# Autodesk Inventor assembly: Assembly1
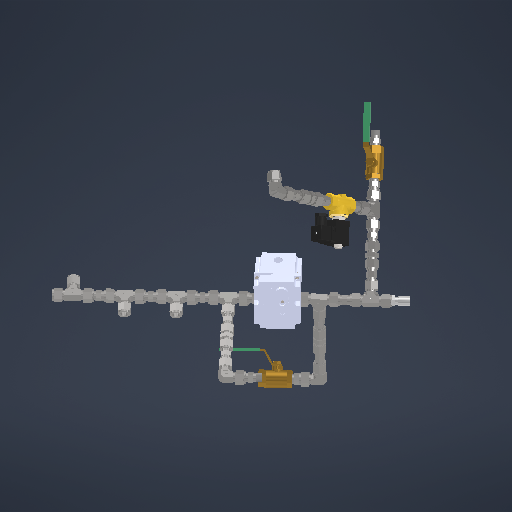
[picture p0: Inventor's stored thumbnail of the model, 512x512]
Saved by Autodesk Inventor 2026.2 (Build 302298000, 298)
## iProperties
Created: 2026-01-25
Part Number: Assembly1
Document SubType Name: Assembly
Designer: szwed
Author: szwed
## Documents named in this file (9)
- C:\Users\szwed\Desktop\R7\Assembly1.iam
- C:\Users\szwed\Documents\Inventor\Content Center Files\R2026\en-US\ISO 49 N8\ISO 49 Hexagon Nipple N8 3_8.ipt
- C:\Users\szwed\Documents\Inventor\Content Center Files\R2026\en-US\Parker A(16)\Parker A-Lok - Fractional Tube 1_2 (4).ipt
- C:\Users\szwed\Documents\Inventor\Content Center Files\R2026\en-US\Parker A(01)\Parker A-Lok - Metric to Inch Tube 12 x 1_2.ipt
- C:\Users\szwed\Documents\Inventor\Content Center Files\R2026\en-US\Parker A-Lok - 90deg Elbow - Fractional Tube\1_2(37).ipt
- C:\Users\szwed\Desktop\gs_solidworks-master\R7_GS_1110_SERVOVALVE\R7_GS_1110_SERVOVALVE\R7_GS_1110_SERVOVALVE\R7_GS_1110_SERVOVALVE.ipt
- C:\Users\szwed\Documents\Inventor\Content Center Files\R2026\en-US\Parker XV500P\Parker Female-Female Pipe Ends XV500P XV500P-8.ipt
- C:\Users\szwed\Documents\Inventor\Content Center Files\R2026\en-US\Parker MTT 2\Parker Male Taper Thread 1_4 x 3_8.ipt
- C:\Users\szwed\Downloads\MV04_DN8_3-8 Zoll\MV04_DN8_3-8 Zoll\MV04_DN8_3-8 Zoll.ipt
## Components (38 placed, 8 different names)
1. ISO 49 Hexagon Nipple N8 3/8:1 — Rigid:1, Rigid:4
2. Parker A-Lok - Fractional Tube 1/2:1 — Rigid:1, Rigid:7, Flush:3
3. ISO 49 Hexagon Nipple N8 3/8:5 — Rigid:5
4. Parker A-Lok - Fractional Tube 1/2:2 — Rigid:4
5. ISO 49 Hexagon Nipple N8 3/8:6 — Rotational:2
6. Parker A-Lok - Fractional Tube 1/2:3 — Rigid:5, Rigid:8, Flush:2
7. ISO 49 Hexagon Nipple N8 3/8:7 — Rigid:7
8. Parker A-Lok - Fractional Tube 1/2:4 — Flush:3
9. Parker A-Lok - Metric to Inch Tube 12 x 1/2:1 — Rotational:1, Rigid:9, Flush:2
10. ISO 49 Hexagon Nipple N8 3/8:8 — Rigid:8, Rotational:1
11. ISO 49 Hexagon Nipple N8 3/8:9 — Rigid:9, Rigid:10
12. Parker A-Lok - 90° Elbow - Fractional Tube 1/2:1 — Rigid:10, Cylindrical:2, Rigid:18
13. R7_GS_1110_SERVOVALVE:1 — Rotational:2, Rotational:3
14. ISO 49 Hexagon Nipple N8 3/8:10 — Rotational:3, Rigid:14
15. Parker A-Lok - Metric to Inch Tube 12 x 1/2:2 — Flush:1
16. ISO 49 Hexagon Nipple N8 3/8:12 — Mate:1, Mate:2, Mate:3
17. ISO 49 Hexagon Nipple N8 3/8:13
18. Parker A-Lok - 90° Elbow - Fractional Tube 1/2:2 — Rigid:16
19. Parker A-Lok - Fractional Tube 1/2:5 — Rigid:14, Mate:1, Rotational:7, Mate:2, Flush:1, Mate:3
20. Parker Female-Female Pipe Ends XV500P XV500P-8:1 — Rigid:17, Cylindrical:1, Rotational:6
21. ISO 49 Hexagon Nipple N8 3/8:14 — Rigid:16, Rigid:17
22. ISO 49 Hexagon Nipple N8 3/8:15 — Cylindrical:1, Cylindrical:2, Rotational:6, Rigid:18
23. ISO 49 Hexagon Nipple N8 3/8:16 — Rotational:7
24. Parker A-Lok - Fractional Tube 1/2:6 — Rotational:8, Rigid:21
25. ISO 49 Hexagon Nipple N8 3/8:17 — Rotational:8, Rotational:9
26. Parker A-Lok - Metric to Inch Tube 12 x 1/2:3 — Rotational:9, Rotational:10
27. ISO 49 Hexagon Nipple N8 3/8:18 — Rotational:10, Rotational:14
28. Parker A-Lok - Fractional Tube 1/2:7 — Rotational:12, Rigid:22, Rotational:14
29. ISO 49 Hexagon Nipple N8 3/8:19 — Rotational:12, Rigid:20
30. Parker Female-Female Pipe Ends XV500P XV500P-8:2 — Rigid:20, Rigid:27
31. Parker Male Taper Thread 1/4 x 3/8:1 — Rigid:21
32. MV04_DN8_3-8 Zoll:1 — Rigid:23, Rigid:24
33. ISO 49 Hexagon Nipple N8 3/8:20 — Rigid:22, Rigid:23
34. ISO 49 Hexagon Nipple N8 3/8:21 — Rigid:24, Rotational:13
35. Parker A-Lok - 90° Elbow - Fractional Tube 1/2:3 — Rigid:26
36. Parker A-Lok - Metric to Inch Tube 12 x 1/2:4 — Rotational:13, Rigid:25
37. ISO 49 Hexagon Nipple N8 3/8:22 — Rigid:25, Rigid:26
38. ISO 49 Hexagon Nipple N8 3/8:23 — Rigid:27
## Relationships (45: WeldJoint 25, RevoluteJoint 12, Mate 3, Flush 3, CylindricalJoint 2)
- Rigid:1 [WeldJoint]: ISO 49 Hexagon Nipple N8 3/8:1 ↔ Parker A-Lok - Fractional Tube 1/2:1
- [WeldJoint]: ISO 49 Hexagon Nipple N8 3/8:5 ↔ Parker A-Lok - Fractional Tube 1/2:2
- [WeldJoint]: ISO 49 Hexagon Nipple N8 3/8:6 ↔ Parker A-Lok - Fractional Tube 1/2:3
- Rigid:4 [WeldJoint]: ISO 49 Hexagon Nipple N8 3/8:1 ↔ Parker A-Lok - Fractional Tube 1/2:2
- Rigid:5 [WeldJoint]: ISO 49 Hexagon Nipple N8 3/8:5 ↔ Parker A-Lok - Fractional Tube 1/2:3
- [WeldJoint]: ISO 49 Hexagon Nipple N8 3/8:7 ↔ Parker A-Lok - Fractional Tube 1/2:4
- Rigid:7 [WeldJoint]: Parker A-Lok - Fractional Tube 1/2:1 ↔ ISO 49 Hexagon Nipple N8 3/8:7
- Rigid:8 [WeldJoint]: Parker A-Lok - Fractional Tube 1/2:3 ↔ ISO 49 Hexagon Nipple N8 3/8:8
- Rotational:1 [RevoluteJoint]: Parker A-Lok - Metric to Inch Tube 12 x 1/2:1 ↔ ISO 49 Hexagon Nipple N8 3/8:8
- Rigid:9 [WeldJoint]: Parker A-Lok - Metric to Inch Tube 12 x 1/2:1 ↔ ISO 49 Hexagon Nipple N8 3/8:9
- Rigid:10 [WeldJoint]: ISO 49 Hexagon Nipple N8 3/8:9 ↔ Parker A-Lok - 90° Elbow - Fractional Tube 1/2:1
- Rotational:2 [RevoluteJoint]: ISO 49 Hexagon Nipple N8 3/8:6 ↔ R7_GS_1110_SERVOVALVE:1
- Rotational:3 [RevoluteJoint]: R7_GS_1110_SERVOVALVE:1 ↔ ISO 49 Hexagon Nipple N8 3/8:10
- [RevoluteJoint]: Parker A-Lok - Metric to Inch Tube 12 x 1/2:2 ↔ ISO 49 Hexagon Nipple N8 3/8:12
- [WeldJoint]: Parker A-Lok - Metric to Inch Tube 12 x 1/2:2 ↔ ISO 49 Hexagon Nipple N8 3/8:13
- [WeldJoint]: ISO 49 Hexagon Nipple N8 3/8:13 ↔ Parker A-Lok - 90° Elbow - Fractional Tube 1/2:2
- Rigid:14 [WeldJoint]: ISO 49 Hexagon Nipple N8 3/8:10 ↔ Parker A-Lok - Fractional Tube 1/2:5
- Rigid:16 [WeldJoint]: Parker A-Lok - 90° Elbow - Fractional Tube 1/2:2 ↔ ISO 49 Hexagon Nipple N8 3/8:14
- Rigid:17 [WeldJoint] (-3 mm): Parker Female-Female Pipe Ends XV500P XV500P-8:1 ↔ ISO 49 Hexagon Nipple N8 3/8:14
- Cylindrical:1: Parker Female-Female Pipe Ends XV500P XV500P-8:1 ↔ ISO 49 Hexagon Nipple N8 3/8:15
- Cylindrical:2: Parker A-Lok - 90° Elbow - Fractional Tube 1/2:1 ↔ ISO 49 Hexagon Nipple N8 3/8:15
- Rotational:6 [RevoluteJoint]: Parker Female-Female Pipe Ends XV500P XV500P-8:1 ↔ ISO 49 Hexagon Nipple N8 3/8:15
- Rigid:18 [WeldJoint]: Parker A-Lok - 90° Elbow - Fractional Tube 1/2:1 ↔ ISO 49 Hexagon Nipple N8 3/8:15
- Mate:1: ISO 49 Hexagon Nipple N8 3/8:12 ↔ Parker A-Lok - Fractional Tube 1/2:5
- [WeldJoint]: ISO 49 Hexagon Nipple N8 3/8:16 ↔ Parker A-Lok - Fractional Tube 1/2:6
- Rotational:7 [RevoluteJoint]: Parker A-Lok - Fractional Tube 1/2:5 ↔ ISO 49 Hexagon Nipple N8 3/8:16
- Mate:2: ISO 49 Hexagon Nipple N8 3/8:12 ↔ Parker A-Lok - Fractional Tube 1/2:5
- Flush:1: Parker A-Lok - Metric to Inch Tube 12 x 1/2:2 ↔ Parker A-Lok - Fractional Tube 1/2:5
- Rotational:8 [RevoluteJoint]: Parker A-Lok - Fractional Tube 1/2:6 ↔ ISO 49 Hexagon Nipple N8 3/8:17
- Rotational:9 [RevoluteJoint]: ISO 49 Hexagon Nipple N8 3/8:17 ↔ Parker A-Lok - Metric to Inch Tube 12 x 1/2:3
- Rotational:10 [RevoluteJoint]: Parker A-Lok - Metric to Inch Tube 12 x 1/2:3 ↔ ISO 49 Hexagon Nipple N8 3/8:18
- Rotational:12 [RevoluteJoint]: Parker A-Lok - Fractional Tube 1/2:7 ↔ ISO 49 Hexagon Nipple N8 3/8:19
- Rigid:20 [WeldJoint]: ISO 49 Hexagon Nipple N8 3/8:19 ↔ Parker Female-Female Pipe Ends XV500P XV500P-8:2
- Rigid:21 [WeldJoint]: Parker A-Lok - Fractional Tube 1/2:6 ↔ Parker Male Taper Thread 1/4 x 3/8:1
- Rigid:22 [WeldJoint]: Parker A-Lok - Fractional Tube 1/2:7 ↔ ISO 49 Hexagon Nipple N8 3/8:20
- Rigid:23 [WeldJoint]: MV04_DN8_3-8 Zoll:1 ↔ ISO 49 Hexagon Nipple N8 3/8:20
- Rigid:24 [WeldJoint]: MV04_DN8_3-8 Zoll:1 ↔ ISO 49 Hexagon Nipple N8 3/8:21
- Rotational:13 [RevoluteJoint]: ISO 49 Hexagon Nipple N8 3/8:21 ↔ Parker A-Lok - Metric to Inch Tube 12 x 1/2:4
- Rigid:25 [WeldJoint]: Parker A-Lok - Metric to Inch Tube 12 x 1/2:4 ↔ ISO 49 Hexagon Nipple N8 3/8:22
- Rigid:26 [WeldJoint]: Parker A-Lok - 90° Elbow - Fractional Tube 1/2:3 ↔ ISO 49 Hexagon Nipple N8 3/8:22
- Rigid:27 [WeldJoint]: Parker Female-Female Pipe Ends XV500P XV500P-8:2 ↔ ISO 49 Hexagon Nipple N8 3/8:23
- Rotational:14 [RevoluteJoint]: ISO 49 Hexagon Nipple N8 3/8:18 ↔ Parker A-Lok - Fractional Tube 1/2:7
- Mate:3: ISO 49 Hexagon Nipple N8 3/8:12 ↔ Parker A-Lok - Fractional Tube 1/2:5
- Flush:2: Parker A-Lok - Fractional Tube 1/2:3 ↔ Parker A-Lok - Metric to Inch Tube 12 x 1/2:1
- Flush:3: Parker A-Lok - Fractional Tube 1/2:1 ↔ Parker A-Lok - Fractional Tube 1/2:4
## Named parameters: d120_d119 = 0 mm, d121_d119 = 0 mm, d124_d119 = 0 mm, d138_d127 = 0 mm, d139_d128 = 132.636605 deg, d140_d129 = 0 mm, d141_d130 = 0 mm, d162_d124_d119 = 0 mm
